# Autodesk Inventor assembly: 케이스 조립
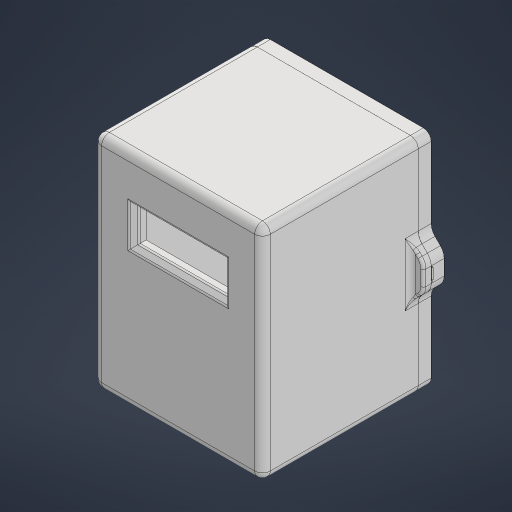
[picture p0: Inventor's stored thumbnail of the model, 512x512]
Saved by Autodesk Inventor 2024 (Build 280153000, 153)
## iProperties
Created: 2023-12-08
Part Number: 케이스 조립
Document SubType Name: Assembly
Designer: KBU
Author: KBU
## Documents named in this file (3)
- C:\Users\KBU\Documents\케이스 조립.iam
- C:\Users\KBU\Documents\케이스 베이스.ipt
- C:\Users\KBU\Documents\케이스 커버.ipt
## Components (2 placed, 2 different names)
1. 케이스 베이스:1 — 삽입:1
2. 케이스 커버:1 — 삽입:1
## Relationships (1: Insert 1)
- 삽입:1 [Insert]: 케이스 베이스:1 ↔ 케이스 커버:1
